# Autodesk Inventor assembly: outer rails
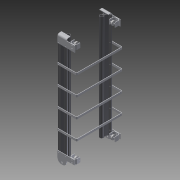
[picture p0: Inventor's stored thumbnail of the model, 180x180]
Saved by Autodesk Inventor 2013 (Build 170138000, 138)
## iProperties
Created: 2013-01-27
Part Number: outer rails
Document SubType Name: Assembly
Designer: Arpan
Author: Arpan
## Documents named in this file (7)
- C:\Users\Arpan\Documents\GitHub\frc2013CAD\Cimber actual\outer rails.iam
- C:\Users\Arpan\Documents\GitHub\frc2013CAD\Cimber actual\Shaft 26 inch.ipt
- C:\Users\Arpan\Documents\GitHub\frc2013CAD\Cimber actual\tie-together tier 2.ipt
- C:\Users\Arpan\Documents\GitHub\frc2013CAD\Cimber actual\endstop.ipt
- C:\Users\Arpan\Documents\GitHub\frc2013CAD\Cimber actual\endstop 2.ipt
- C:\Users\Arpan\Documents\GitHub\frc2013CAD\Cimber actual\arm mout.ipt
- C:\Users\Arpan\Documents\GitHub\frc2013CAD\Cimber actual\mini pulley assembly.iam
## Components (14 placed, 6 different names)
1. Shaft 26 inch:1 — Angle:1, Flush:1, Mate:5, Mate:6, Mate:7, Mate:8, Mate:9, Mate:10, Mate:11, Mate:12, Mate:14, Mate:24, Mate:25, Mate:26, Mate:30, Mate:31, Mate:32
2. Shaft 26 inch:2 — Angle:1, Flush:1, Mate:2, Angle:2, Mate:3, Mate:13, Mate:16, Mate:17, Mate:21, Mate:22, Mate:23, Mate:27, Mate:28, Mate:29, Mate:33, Mate:40
3. tie-together tier 2:1 — Mate:2, Angle:2, Mate:3, Mate:5, Mate:6, Mate:33
4. tie-together tier 2:2 — Mate:7, Mate:8, Mate:9
5. tie-together tier 2:3 — Mate:10, Mate:11, Mate:12, Mate:13, Mate:40
6. tie-together tier 2:4 — Mate:14, Mate:16, Mate:17
7. endstop:1 — Mate:24, Mate:25, Mate:26, Mate:37, Flush:3, Flush:4
8. endstop 2:1 — Mate:21, Mate:22, Mate:23, Mate:34, Flush:2, Mate:35, Mate:36
9. arm mout:2 — Mate:27, Mate:28, Mate:29, Mate:38, Flush:5, Flush:6
10. arm mout:3 — Mate:30, Mate:31, Mate:32, Mate:39, Flush:7, Flush:8
11. mini pulley assembly:1 [sub-assembly] — Mate:39, Flush:7, Flush:8
12. mini pulley assembly:2 [sub-assembly] — Mate:38, Flush:5, Flush:6
13. mini pulley assembly:3 [sub-assembly] — Mate:34, Flush:2, Mate:35, Mate:36
14. mini pulley assembly:4 [sub-assembly] — Mate:37, Flush:3, Flush:4
## Relationships (44: Mate 34, Flush 8, Angle 2)
- Angle:1 (180 deg): Shaft 26 inch:1 ↔ Shaft 26 inch:2
- Flush:1: Shaft 26 inch:1 ↔ Shaft 26 inch:2
- Mate:2: Shaft 26 inch:2 ↔ tie-together tier 2:1
- Angle:2 (0 deg): Shaft 26 inch:2 ↔ tie-together tier 2:1
- Mate:3: Shaft 26 inch:2 ↔ tie-together tier 2:1
- Mate:5: Shaft 26 inch:1 ↔ tie-together tier 2:1
- Mate:6: Shaft 26 inch:1 ↔ tie-together tier 2:1
- Mate:7: Shaft 26 inch:1 ↔ tie-together tier 2:2
- Mate:8: Shaft 26 inch:1 ↔ tie-together tier 2:2
- Mate:9: Shaft 26 inch:1 ↔ tie-together tier 2:2
- Mate:10: Shaft 26 inch:1 ↔ tie-together tier 2:3
- Mate:11: Shaft 26 inch:1 ↔ tie-together tier 2:3
- Mate:12: Shaft 26 inch:1 ↔ tie-together tier 2:3
- Mate:13: Shaft 26 inch:2 ↔ tie-together tier 2:3
- Mate:14: Shaft 26 inch:1 ↔ tie-together tier 2:4
- Mate:16: Shaft 26 inch:2 ↔ tie-together tier 2:4
- Mate:17: Shaft 26 inch:2 ↔ tie-together tier 2:4
- Mate:21: Shaft 26 inch:2 ↔ endstop 2:1
- Mate:22: Shaft 26 inch:2 ↔ endstop 2:1
- Mate:23: Shaft 26 inch:2 ↔ endstop 2:1
- Mate:24: Shaft 26 inch:1 ↔ endstop:1
- Mate:25: Shaft 26 inch:1 ↔ endstop:1
- Mate:26: Shaft 26 inch:1 ↔ endstop:1
- Mate:27: Shaft 26 inch:2 ↔ arm mout:2
- Mate:28: Shaft 26 inch:2 ↔ arm mout:2
- Mate:29: Shaft 26 inch:2 ↔ arm mout:2
- Mate:30: Shaft 26 inch:1 ↔ arm mout:3
- Mate:31: Shaft 26 inch:1 ↔ arm mout:3
- Mate:32: Shaft 26 inch:1 ↔ arm mout:3
- Mate:33: Shaft 26 inch:2 ↔ tie-together tier 2:1
- Mate:34: endstop 2:1 ↔ mini pulley assembly:3
- Flush:2: endstop 2:1 ↔ mini pulley assembly:3
- Mate:35: endstop 2:1 ↔ mini pulley assembly:3
- Mate:36: endstop 2:1 ↔ mini pulley assembly:3
- Mate:37: endstop:1 ↔ mini pulley assembly:4
- Flush:3: endstop:1 ↔ mini pulley assembly:4
- Flush:4: endstop:1 ↔ mini pulley assembly:4
- Mate:38: arm mout:2 ↔ mini pulley assembly:2
- Flush:5: arm mout:2 ↔ mini pulley assembly:2
- Flush:6: arm mout:2 ↔ mini pulley assembly:2
- Mate:39: arm mout:3 ↔ mini pulley assembly:1
- Flush:7: arm mout:3 ↔ mini pulley assembly:1
- Flush:8: arm mout:3 ↔ mini pulley assembly:1
- Mate:40: Shaft 26 inch:2 ↔ tie-together tier 2:3
